# Autodesk Inventor assembly: 6 HiGrip with bearings, pulleys and spacers
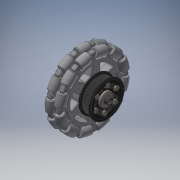
[picture p0: Inventor's stored thumbnail of the model, 180x180]
Saved by Autodesk Inventor 2018 (Build 220112000, 112)
## iProperties
Created: 2020-01-29
Part Number: 6 HiGrip with bearings, pulleys and spacers
Document SubType Name: Assembly
Designer: Weeb No1
Author: Weeb No1
## Documents named in this file (9)
- \\studenthome\students\S-2512711\GitHub\2020CAD\Gabriel Inventor Files (Shooter, Drivebase)\Drivebase Assembly\Part Files\6 Omni with bearings, pulleys and spacers.iam
- \\studenthome\students\S-2512711\GitHub\2020CAD\Gabriel Inventor Files (Shooter, Drivebase)\Drivebase Assembly\Part Files\42 tooth HTD Pulley half 2014.ipt
- \\studenthome\students\S-2512711\GitHub\2020CAD\Gabriel Inventor Files (Shooter, Drivebase)\Drivebase Assembly\Part Files\1614Z Bearing.ipt
- \\studenthome\students\S-2512711\GitHub\2020CAD\Gabriel Inventor Files (Shooter, Drivebase)\Drivebase Assembly\Part Files\10-24 Hex Washer Rolling x 1.ipt
- \\studenthome\students\S-2512711\GitHub\2020CAD\Gabriel Inventor Files (Shooter, Drivebase)\Drivebase Assembly\Part Files\am-1306 spacer 0280 WashersUSA 13RS052001.ipt
- \\studenthome\students\S-2512711\GitHub\2020CAD\Gabriel Inventor Files (Shooter, Drivebase)\Drivebase Assembly\Part Files\6_Omni-Directional_Wheel_217-2585.iam
- \\studenthome\students\S-2512711\GitHub\2020CAD\Gabriel Inventor Files (Shooter, Drivebase)\Drivebase Assembly\Part Files\0_375_ID_x_1_125_OD_x_0_313_WD_Flanged_Bearing_217-2732.ipt
- \\studenthome\students\S-2512711\GitHub\2020CAD\Gabriel Inventor Files (Shooter, Drivebase)\Drivebase Assembly\Part Files\Omni wheel spacer.ipt
- \\studenthome\students\S-2512711\GitHub\2020CAD\Gabriel Inventor Files (Shooter, Drivebase)\Drivebase Assembly\Part Files\Omni wheel spacer 2.ipt
## Components (15 placed, 8 different names)
1. 42 tooth HTD Pulley half 2014:1 — Mate:2, Mate:3, Mate:4, Mate:26, Rotation:3, Rotation:4
2. 42 tooth HTD Pulley half 2014:2 — Mate:1, Mate:2, Mate:3, Mate:4, Mate:5, Mate:8, Mate:9, Mate:10, Mate:11, Mate:12, Mate:13, Mate:14, Mate:15, Mate:16, Mate:17, Mate:18, Mate:19, Rotation:2, Rotation:3
3. 1614Z Bearing:1 — Mate:1, Mate:5, Mate:6, Mate:7, Rotation:1, Rotation:2, Mate:29, Mate:30
4. 10-24 Hex Washer Rolling x 1:1 — Mate:12, Mate:17, Mate:25
5. 10-24 Hex Washer Rolling x 1:2 — Mate:9, Mate:18, Mate:24
6. 10-24 Hex Washer Rolling x 1:3 — Mate:11, Mate:15
7. 10-24 Hex Washer Rolling x 1:4 — Mate:10, Mate:16
8. 10-24 Hex Washer Rolling x 1:5 — Mate:8, Mate:19
9. 10-24 Hex Washer Rolling x 1:6 — Mate:13, Mate:14
10. am-1306 spacer 0280 WashersUSA 13RS052001:1 — Mate:6, Mate:7, Rotation:1
11. Omni wheel spacer 2:1 — Mate:27, Mate:28, Rotation:8
12. 6_Omni-Directional_Wheel_217-2585:1 [sub-assembly] — Mate:20, Mate:21, Mate:22, Mate:23, Mate:24, Mate:25, Mate:26, Rotation:4
13. 0_375_ID_x_1_125_OD_x_0_313_WD_Flanged_Bearing_217-2732:1 — Mate:20, Mate:21, Mate:27, Mate:28, Rotation:8
14. 0_375_ID_x_1_125_OD_x_0_313_WD_Flanged_Bearing_217-2732:2 — Mate:22, Mate:23, Rotation:7
15. Omni wheel spacer:1 — Mate:29, Mate:30, Rotation:7
## Relationships (36: Mate 30, RelateRotation 6)
- Mate:1: 42 tooth HTD Pulley half 2014:2 ↔ 1614Z Bearing:1
- Mate:2: 42 tooth HTD Pulley half 2014:1 ↔ 42 tooth HTD Pulley half 2014:2
- Mate:3: 42 tooth HTD Pulley half 2014:1 ↔ 42 tooth HTD Pulley half 2014:2
- Mate:4: 42 tooth HTD Pulley half 2014:1 ↔ 42 tooth HTD Pulley half 2014:2
- Mate:5: 42 tooth HTD Pulley half 2014:2 ↔ 1614Z Bearing:1
- Mate:6: 1614Z Bearing:1 ↔ am-1306 spacer 0280 WashersUSA 13RS052001:1
- Mate:7: 1614Z Bearing:1 ↔ am-1306 spacer 0280 WashersUSA 13RS052001:1
- Mate:8: 42 tooth HTD Pulley half 2014:2 ↔ 10-24 Hex Washer Rolling x 1:5
- Mate:9: 42 tooth HTD Pulley half 2014:2 ↔ 10-24 Hex Washer Rolling x 1:2
- Mate:10: 42 tooth HTD Pulley half 2014:2 ↔ 10-24 Hex Washer Rolling x 1:4
- Mate:11: 42 tooth HTD Pulley half 2014:2 ↔ 10-24 Hex Washer Rolling x 1:3
- Mate:12: 42 tooth HTD Pulley half 2014:2 ↔ 10-24 Hex Washer Rolling x 1:1
- Mate:13: 42 tooth HTD Pulley half 2014:2 ↔ 10-24 Hex Washer Rolling x 1:6
- Mate:14: 42 tooth HTD Pulley half 2014:2 ↔ 10-24 Hex Washer Rolling x 1:6
- Mate:15: 42 tooth HTD Pulley half 2014:2 ↔ 10-24 Hex Washer Rolling x 1:3
- Mate:16: 42 tooth HTD Pulley half 2014:2 ↔ 10-24 Hex Washer Rolling x 1:4
- Mate:17: 42 tooth HTD Pulley half 2014:2 ↔ 10-24 Hex Washer Rolling x 1:1
- Mate:18: 42 tooth HTD Pulley half 2014:2 ↔ 10-24 Hex Washer Rolling x 1:2
- Mate:19: 42 tooth HTD Pulley half 2014:2 ↔ 10-24 Hex Washer Rolling x 1:5
- Mate:20: 6_Omni-Directional_Wheel_217-2585:1 ↔ 0_375_ID_x_1_125_OD_x_0_313_WD_Flanged_Bearing_217-2732:1
- Mate:21: 6_Omni-Directional_Wheel_217-2585:1 ↔ 0_375_ID_x_1_125_OD_x_0_313_WD_Flanged_Bearing_217-2732:1
- Mate:22: 6_Omni-Directional_Wheel_217-2585:1 ↔ 0_375_ID_x_1_125_OD_x_0_313_WD_Flanged_Bearing_217-2732:2
- Mate:23: 6_Omni-Directional_Wheel_217-2585:1 ↔ 0_375_ID_x_1_125_OD_x_0_313_WD_Flanged_Bearing_217-2732:2
- Mate:24: 10-24 Hex Washer Rolling x 1:2 ↔ 6_Omni-Directional_Wheel_217-2585:1
- Mate:25: 10-24 Hex Washer Rolling x 1:1 ↔ 6_Omni-Directional_Wheel_217-2585:1
- Mate:26 (1.5875 mm): 42 tooth HTD Pulley half 2014:1 ↔ 6_Omni-Directional_Wheel_217-2585:1
- Mate:27: Omni wheel spacer 2:1 ↔ 0_375_ID_x_1_125_OD_x_0_313_WD_Flanged_Bearing_217-2732:1
- Mate:28: Omni wheel spacer 2:1 ↔ 0_375_ID_x_1_125_OD_x_0_313_WD_Flanged_Bearing_217-2732:1
- Rotation:1 [RelateRotation] (1 ul): 1614Z Bearing:1 ↔ am-1306 spacer 0280 WashersUSA 13RS052001:1
- Rotation:2 [RelateRotation] (1 ul): 42 tooth HTD Pulley half 2014:2 ↔ 1614Z Bearing:1
- Rotation:3 [RelateRotation] (1 ul): 42 tooth HTD Pulley half 2014:1 ↔ 42 tooth HTD Pulley half 2014:2
- Rotation:4 [RelateRotation] (1 ul): 42 tooth HTD Pulley half 2014:1 ↔ 6_Omni-Directional_Wheel_217-2585:1
- Mate:29: 1614Z Bearing:1 ↔ Omni wheel spacer:1
- Mate:30: 1614Z Bearing:1 ↔ Omni wheel spacer:1
- Rotation:7 [RelateRotation] (2 ul): 0_375_ID_x_1_125_OD_x_0_313_WD_Flanged_Bearing_217-2732:2 ↔ Omni wheel spacer:1
- Rotation:8 [RelateRotation] (1 ul): Omni wheel spacer 2:1 ↔ 0_375_ID_x_1_125_OD_x_0_313_WD_Flanged_Bearing_217-2732:1
